# Autodesk Inventor assembly: Plataforma_flotante
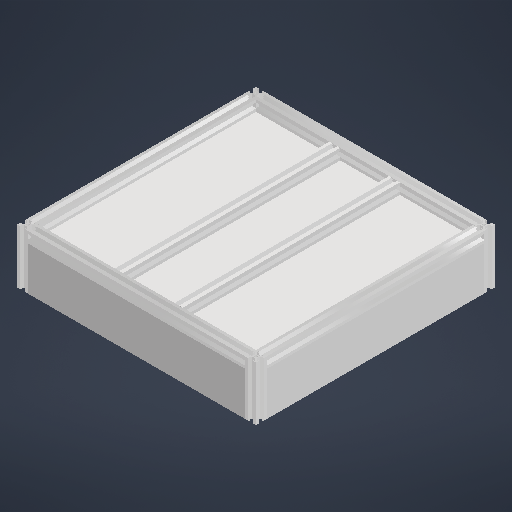
[picture p0: Inventor's stored thumbnail of the model, 512x512]
Saved by Autodesk Inventor 2026 (Build 300175050, 175E)
## iProperties
Created: 2024-02-07
Part Number: Plataforma_flotante
Document SubType Name: Assembly
Designer: diego
Mass: 53763.4 g
Surface Area: 46869.6 cm^2
Volume: 53763.4 cm^3
Author: diego
## Documents named in this file (5)
- C:\Users\habbo\OneDrive\Documents\UTEC\2025-2\Mecanismo\Plataforma_validacion (1)\Plataforma_validacion\Plataforma_flotante\Plataforma_flotante.iam
- C:\Users\habbo\OneDrive\Documents\UTEC\2025-2\Mecanismo\Plataforma_validacion (1)\Plataforma_validacion\Plataforma_flotante\vslot_400mm.ipt
- C:\Users\habbo\OneDrive\Documents\UTEC\2025-2\Mecanismo\Plataforma_validacion (1)\Plataforma_validacion\Plataforma_flotante\vslot_100mm.ipt
- C:\Users\habbo\OneDrive\Documents\UTEC\2025-2\Mecanismo\Plataforma_validacion (1)\Plataforma_validacion\Plataforma_flotante\Tapa base.ipt
- C:\Users\habbo\OneDrive\Documents\UTEC\2025-2\Mecanismo\Plataforma_validacion (1)\Plataforma_validacion\Plataforma_flotante\Tapa lados.ipt
## Components (15 placed, 4 different names)
1. vslot_100mm:1 — Mate:43, Flush:62, Flush:66, Flush:67, Mate:53
2. vslot_400mm:2 — Mate:41
3. vslot_400mm:1 — Mate:42, Flush:61, Mate:46, Mate:54
4. vslot_100mm:3 — Flush:63, Flush:64, Mate:50
5. vslot_100mm:4 — Flush:65, Mate:52
6. vslot_400mm:4 — Mate:40, Mate:49
7. vslot_400mm:3 — Mate:51
8. vslot_100mm:5
9. Tapa base:1 — Mate:40, Mate:41, Mate:42, Mate:44, Mate:45
10. Tapa lados:1 — Flush:61, Mate:43, Flush:62
11. vslot_400mm:5 — Mate:44, Mate:46, Mate:48, Mate:49
12. vslot_400mm:6 — Mate:45, Mate:48, Mate:54
13. Tapa lados:2 — Flush:65, Mate:51, Mate:52
14. Tapa lados:3 — Flush:66, Flush:67, Mate:53
15. Tapa lados:4 — Flush:63, Flush:64, Mate:50
## Relationships (42: Mate 21, Flush 21)
- [Mate]: vslot_100mm:1 ↔ vslot_400mm:2
- [Mate]: vslot_100mm:1 ↔ vslot_400mm:1
- [Flush]: vslot_400mm:2 ↔ vslot_400mm:1
- [Flush]: vslot_100mm:1 ↔ vslot_400mm:1
- [Flush]: vslot_100mm:1 ↔ vslot_400mm:2
- [Flush]: vslot_100mm:1 ↔ vslot_400mm:2
- [Mate]: vslot_400mm:1 ↔ vslot_100mm:3
- [Flush]: vslot_400mm:1 ↔ vslot_100mm:3
- [Flush]: vslot_400mm:1 ↔ vslot_100mm:3
- [Mate]: vslot_100mm:4 ↔ vslot_400mm:4
- [Mate]: vslot_100mm:4 ↔ vslot_400mm:3
- [Flush]: vslot_400mm:4 ↔ vslot_400mm:3
- [Flush]: vslot_100mm:4 ↔ vslot_400mm:3
- [Flush]: vslot_100mm:4 ↔ vslot_400mm:4
- [Flush]: vslot_100mm:4 ↔ vslot_400mm:4
- [Mate]: vslot_400mm:3 ↔ vslot_100mm:5
- [Flush]: vslot_400mm:3 ↔ vslot_100mm:5
- [Flush]: vslot_400mm:3 ↔ vslot_100mm:5
- [Mate]: vslot_400mm:2 ↔ vslot_100mm:5
- [Flush]: vslot_400mm:2 ↔ vslot_100mm:4
- [Flush]: vslot_400mm:2 ↔ vslot_100mm:5
- Mate:40: vslot_400mm:4 ↔ Tapa base:1
- Mate:41: vslot_400mm:2 ↔ Tapa base:1
- Mate:42: vslot_400mm:1 ↔ Tapa base:1
- Flush:61: vslot_400mm:1 ↔ Tapa lados:1
- Mate:43: vslot_100mm:1 ↔ Tapa lados:1
- Flush:62: vslot_100mm:1 ↔ Tapa lados:1
- Mate:44: Tapa base:1 ↔ vslot_400mm:5
- Mate:45: Tapa base:1 ↔ vslot_400mm:6
- Mate:46: vslot_400mm:1 ↔ vslot_400mm:5
- Mate:48 (90 mm): vslot_400mm:5 ↔ vslot_400mm:6
- Mate:49 (135 mm): vslot_400mm:4 ↔ vslot_400mm:5
- Flush:63: vslot_100mm:3 ↔ Tapa lados:4
- Flush:64: vslot_100mm:3 ↔ Tapa lados:4
- Mate:50: vslot_100mm:3 ↔ Tapa lados:4
- Flush:65: vslot_100mm:4 ↔ Tapa lados:2
- Mate:51: vslot_400mm:3 ↔ Tapa lados:2
- Mate:52: vslot_100mm:4 ↔ Tapa lados:2
- Flush:66: vslot_100mm:1 ↔ Tapa lados:3
- Flush:67: vslot_100mm:1 ↔ Tapa lados:3
- Mate:53: vslot_100mm:1 ↔ Tapa lados:3
- Mate:54: vslot_400mm:1 ↔ vslot_400mm:6
## Named parameters: d456_d444 = 0 mm, d457_d445 = 0 mm, d458_d446 = 0 mm, d459_d392 = 0 mm, d460_d393 = 0 mm, d461_d394 = 0 mm, d462_d395 = 0 mm, d478_d390 = 0 mm, d479_d391 = 0 mm
